# Autodesk Inventor assembly: IN-12_Nixie_Board
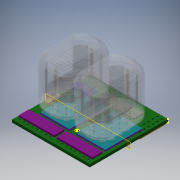
[picture p0: Inventor's stored thumbnail of the model, 180x180]
Saved by Autodesk Inventor 2019 (Build 230136000, 136)
## iProperties
Created: 2019-08-02
Part Number: IN-12_Nixie_Board
Material: Generisch
Document SubType Name: Assembly
Designer: grubi
Author: grubi
## Documents named in this file (3)
- \\diskstation\home\NixieBaugruppe\IN-12_Nixie_Board.iam
- \\diskstation\home\NixieBaugruppe\NixieModule_IN12.brd.ipt
- \\diskstation\home\idf\IN-12\IN-12a.ipt
## Components (3 placed, 2 different names)
1. IN-12a:2 — Fluchtend:1, Fluchtend:2, Passend:2
2. IN-12a:1 — Fluchtend:1, Fluchtend:2, Passend:1, Passend:3
3. NixieModule_IN12.brd:1 — Passend:1, Passend:2, Passend:3
## Relationships (5: Mate 3, Flush 2)
- Fluchtend:1 [Flush]: IN-12a:2 ↔ IN-12a:1
- Fluchtend:2 [Flush]: IN-12a:2 ↔ IN-12a:1
- Passend:1 [Mate] (-34 mm): IN-12a:1 ↔ NixieModule_IN12.brd:1
- Passend:2 [Mate]: IN-12a:2 ↔ NixieModule_IN12.brd:1
- Passend:3 [Mate]: IN-12a:1 ↔ NixieModule_IN12.brd:1
